# Autodesk Inventor assembly: rbc support
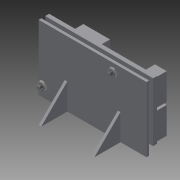
[picture p0: Inventor's stored thumbnail of the model, 180x180]
Saved by Autodesk Inventor 2015 (Build 190159000, 159)
## iProperties
Created: 2015-05-04
Part Number: rbc support
Document SubType Name: Assembly
Designer: Kuba
Author: Kuba
## Documents named in this file (6)
- C:\Users\Kuba\Dysk Google\synergia\Synergolf\model\GOLF\rbc support\rbc support.iam
- C:\Users\Kuba\Dysk Google\synergia\Synergolf\model\GOLF\RBC4242.ipt
- C:\Users\Kuba\Dysk Google\synergia\Synergolf\model\GOLF\rbc support\blacha pion rbc.ipt
- C:\Users\Kuba\Dysk Google\synergia\Synergolf\model\GOLF\driver\wspornik.ipt
- C:\Users\Kuba\Dysk Google\synergia\Synergolf\model\GOLF\ContentCenter\pl-PL\DIN 912\DIN 912 - M3 x 0,5 x 12 x 10,75.ipt
- C:\Users\Kuba\Dysk Google\synergia\Synergolf\model\GOLF\ContentCenter\pl-PL\DIN 439-2\DIN 439 - M3 x 0,5.ipt
## Components (8 placed, 5 different names)
1. RBC4242:1 — Zestawiający:1, Równoległy:1, Równoległy:2, Zestawiający:3, Zestawiający:4, Zestawiający:5, Zestawiający:6
2. blacha pion rbc:1 — Zestawiający:1, Równoległy:1, Równoległy:2, Zestawiający:2, Równoległy:3, Równoległy:4, Wstaw:1, Wstaw:2
3. DIN 912 - zastąpiona przez DIN EN ISO 4762 M3 x 12:1 — Zestawiający:3, Zestawiający:4
4. DIN 912 - zastąpiona przez DIN EN ISO 4762 M3 x 12:2 — Zestawiający:5, Zestawiający:6
5. DIN 439-2 - zastąpiona przez DIN EN 24035/28675 M3:1 — Wstaw:1
6. DIN 439-2 - zastąpiona przez DIN EN 24035/28675 M3:2 — Wstaw:2
7. wspornik:1 — Zestawiający:2, Równoległy:3, Równoległy:4
8. wspornik:2
## Component patterns: (2 elements, first: wspornik:1)
## Relationships (12: Mate 6, Flush 4, Insert 2)
- Zestawiający:1 [Mate] (3 mm): RBC4242:1 ↔ blacha pion rbc:1
- Równoległy:1 [Flush]: RBC4242:1 ↔ blacha pion rbc:1
- Równoległy:2 [Flush]: RBC4242:1 ↔ blacha pion rbc:1
- Zestawiający:2 [Mate]: blacha pion rbc:1 ↔ wspornik:1
- Równoległy:3 [Flush]: blacha pion rbc:1 ↔ wspornik:1
- Równoległy:4 [Flush] (20 mm): blacha pion rbc:1 ↔ wspornik:1
- Zestawiający:3 [Mate]: RBC4242:1 ↔ DIN 912 - zastąpiona przez DIN EN ISO 4762 M3 x 12:1
- Zestawiający:4 [Mate]: RBC4242:1 ↔ DIN 912 - zastąpiona przez DIN EN ISO 4762 M3 x 12:1
- Zestawiający:5 [Mate]: RBC4242:1 ↔ DIN 912 - zastąpiona przez DIN EN ISO 4762 M3 x 12:2
- Zestawiający:6 [Mate]: RBC4242:1 ↔ DIN 912 - zastąpiona przez DIN EN ISO 4762 M3 x 12:2
- Wstaw:1 [Insert]: blacha pion rbc:1 ↔ DIN 439-2 - zastąpiona przez DIN EN 24035/28675 M3:1
- Wstaw:2 [Insert]: blacha pion rbc:1 ↔ DIN 439-2 - zastąpiona przez DIN EN 24035/28675 M3:2
